# Autodesk Inventor assembly: BBM Assembly
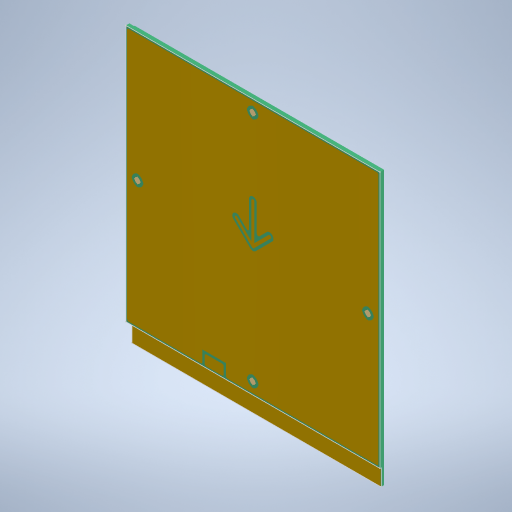
[picture p0: Inventor's stored thumbnail of the model, 512x512]
Saved by Autodesk Inventor 2023 (Build 270158000, 158)
## iProperties
Created: 2022-05-02
Part Number: BBM Assembly
Document SubType Name: Assembly
Designer: Caleb
Author: Caleb
## Documents named in this file (3)
- C:\Users\Caleb\Desktop\nebraska-silicon-lab\Hardware\ETL\modules\throughput mockups\BBM Assembly.iam
- C:\Users\Caleb\Desktop\nebraska-silicon-lab\Hardware\ETL\modules\throughput mockups\etl_lgad_mockup_v1p1.ipt
- C:\Users\Caleb\Desktop\nebraska-silicon-lab\Hardware\ETL\modules\throughput mockups\etl_etroc_mockup_v1p1.ipt
## Components (2 placed, 2 different names)
1. etl_lgad_mockup_v1p1:1 — Mate:1, Angle:1, Flush:1, Flush:2
2. etl_etroc_mockup_v1p1:1 — Mate:1, Angle:1, Flush:1, Flush:2
## Relationships (4: Flush 2, Mate 1, Angle 1)
- Mate:1: etl_lgad_mockup_v1p1:1 ↔ etl_etroc_mockup_v1p1:1
- Angle:1 (0 deg): etl_lgad_mockup_v1p1:1 ↔ etl_etroc_mockup_v1p1:1
- Flush:1 (-0.2 mm): etl_lgad_mockup_v1p1:1 ↔ etl_etroc_mockup_v1p1:1
- Flush:2 (-0.2 mm): etl_lgad_mockup_v1p1:1 ↔ etl_etroc_mockup_v1p1:1
